# Autodesk Inventor assembly: booth
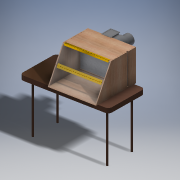
[picture p0: Inventor's stored thumbnail of the model, 180x180]
Saved by Autodesk Inventor 2017 (Build 210142000, 142)
## iProperties
Created: 2019-04-11
Part Number: booth
Document SubType Name: Assembly
Designer: Brian
Author: Brian
## Documents named in this file (24)
- B:\Miniatures\spray booth\large 26-inch, rightangled back\booth.iam
- B:\Miniatures\spray booth\large 26-inch, rightangled back\Frame - Horizontal (Bottom Front).ipt
- B:\Miniatures\spray booth\large 26-inch, rightangled back\Frame - Horizontal (Bottom Rear).ipt
- B:\Miniatures\spray booth\large 26-inch, rightangled back\Frame - Horizontal (Top Front).ipt
- B:\Miniatures\spray booth\large 26-inch, rightangled back\Frame - Horizontal (Top Rear).ipt
- B:\Miniatures\spray booth\large 26-inch, rightangled back\Back Side.ipt
- B:\Miniatures\spray booth\large 26-inch, rightangled back\Cap Side.ipt
- B:\Miniatures\spray booth\large 26-inch, rightangled back\Frame - Vertical (Clones).ipt
- B:\Miniatures\spray booth\large 26-inch, rightangled back\Frame - Vertical (Left Front).ipt
- B:\Miniatures\spray booth\large 26-inch, rightangled back\Two By Four - Rectangle.ipt
- B:\Miniatures\spray booth\large 26-inch, rightangled back\Top Side.ipt
- B:\Miniatures\spray booth\large 26-inch, rightangled back\Left Side.ipt
- B:\Miniatures\spray booth\large 26-inch, rightangled back\Bottom Base.ipt
- B:\Miniatures\spray booth\large 26-inch, rightangled back\Right Side - Rear.ipt
- B:\Miniatures\spray booth\large 26-inch, rightangled back\Right Side - Forward.ipt
- B:\Miniatures\spray booth\large 26-inch, rightangled back\Filter.ipt
- B:\Miniatures\spray booth\large 26-inch, rightangled back\Acrylic Panel - Top.ipt
- B:\Miniatures\spray booth\large 26-inch, rightangled back\Acrylic Panel - Bottom.ipt
- B:\Miniatures\spray booth\large 26-inch, rightangled back\PianoHingePlate.ipt
- B:\Miniatures\spray booth\large 26-inch, rightangled back\PianoHingePin.ipt
- B:\Miniatures\spray booth\large 26-inch, rightangled back\dayton1TDT2 $167.ipt
- B:\Miniatures\spray booth\large 26-inch, rightangled back\table.ipt
- B:\Miniatures\spray booth\textures\Wrinkled Paper.jpg
- B:\Miniatures\spray booth\textures\images.png
## Components (25 placed, 21 different names)
1. Frame - Horizontal (Bottom Front):1 — Slider:1
2. Frame - Horizontal (Bottom Rear):1
3. Frame - Horizontal (Top Front):1
4. Frame - Horizontal (Top Rear):1
5. Back Side:1 — Mate:16
6. Cap Side:1 — Flush:4, Mate:14
7. Frame - Vertical (Clones):1
8. Frame - Vertical (Left Front):1
9. Two By Four - Rectangle:1
10. Top Side:1 — Mate:15, Flush:7
11. Left Side:1 — Flush:8
12. Bottom Base:1 — Slider:2
13. Right Side - Forward:1 — Flush:9
14. Right Side - Rear:1
15. Filter:1 — Slider:1
16. Acrylic Panel - Top:1 — Flush:1, Mate:7, Mate:8, Mate:10, Flush:2, Mate:11
17. Acrylic Panel - Bottom:1 — Mate:12, Flush:3, Mate:13
18. PianoHingePlate:1 — Flush:1, Mate:7, Mate:8, Rotational:1, Insert:1
19. PianoHingePlate:2 — Rotational:1, Mate:14, Mate:15, Flush:9
20. PianoHingePin:1 — Insert:1
21. PianoHingePlate:3 — Mate:10, Flush:2, Mate:11, Rotational:2, Insert:2
22. PianoHingePlate:4 — Rotational:2, Mate:12, Flush:3, Mate:13
23. PianoHingePin:2 — Insert:2
24. dayton1TDT2 $167:2 — Flush:4, Mate:16, Flush:7, Flush:8
25. table:1 — Slider:2
## Relationships (22: Mate 9, Flush 7, TranslationJoint 2, RevoluteJoint 2, Insert 2)
- Slider:1 [TranslationJoint]: Frame - Horizontal (Bottom Front):1 ↔ Filter:1
- Flush:1 (25.4 mm): Acrylic Panel - Top:1 ↔ PianoHingePlate:1
- Mate:7: Acrylic Panel - Top:1 ↔ PianoHingePlate:1
- Mate:8: Acrylic Panel - Top:1 ↔ PianoHingePlate:1
- Rotational:1 [RevoluteJoint]: PianoHingePlate:1 ↔ PianoHingePlate:2
- Insert:1: PianoHingePlate:1 ↔ PianoHingePin:1
- Mate:10: Acrylic Panel - Top:1 ↔ PianoHingePlate:3
- Flush:2 (25.4 mm): Acrylic Panel - Top:1 ↔ PianoHingePlate:3
- Mate:11: Acrylic Panel - Top:1 ↔ PianoHingePlate:3
- Rotational:2 [RevoluteJoint]: PianoHingePlate:3 ↔ PianoHingePlate:4
- Mate:12: Acrylic Panel - Bottom:1 ↔ PianoHingePlate:4
- Flush:3 (25.4 mm): Acrylic Panel - Bottom:1 ↔ PianoHingePlate:4
- Mate:13: Acrylic Panel - Bottom:1 ↔ PianoHingePlate:4
- Insert:2: PianoHingePlate:3 ↔ PianoHingePin:2
- Slider:2 [TranslationJoint]: Bottom Base:1 ↔ table:1
- Flush:4: Cap Side:1 ↔ dayton1TDT2 $167:2
- Mate:14: Cap Side:1 ↔ PianoHingePlate:2
- Mate:15 (393.7 mm): Top Side:1 ↔ PianoHingePlate:2
- Mate:16: Back Side:1 ↔ dayton1TDT2 $167:2
- Flush:7: Top Side:1 ↔ dayton1TDT2 $167:2
- Flush:8 (203.2 mm): Left Side:1 ↔ dayton1TDT2 $167:2
- Flush:9 (25.4 mm): Right Side - Forward:1 ↔ PianoHingePlate:2
